# Autodesk Inventor assembly: Drive Roller Assembly 3 (Lexan)
(part 2 of 2)
- Mate:1086: Vex Pro 1x1 rectangular tubing 2 in length:2 ↔ Vex Pro 90 degree gusset (1-8 in):3
- Mate:1087: Spacer 2:4 ↔ Vex Pro 90 degree gusset (1-8 in):3
- Mate:1088: Spacer 2:4 ↔ Vex Pro 90 degree gusset (1-8 in):3
- Mate:1090: Vex Pro 1x1 rectangular tubing 2 in length:4 ↔ Vex Pro 90 degree gusset (1-8 in):4
- Mate:1091: Vex Pro 1x1 rectangular tubing 2 in length:4 ↔ Vex Pro 90 degree gusset (1-8 in):4
- Mate:1092: Vex Pro 1x1 rectangular tubing 14 in length:6 ↔ Vex Pro 90 degree gusset (1-8 in):4
- Mate:1093: Spacer 2:3 ↔ Vex Pro 90 degree gusset (1-8 in):4
- Mate:1094: Spacer 2:6 ↔ Vex Pro 90 degree gusset (1-8 in):4
- Mate:1096: Spacer 2:6 ↔ Vex Pro 90 degree gusset (1-8 in):4
- Mate:1100: Clamp with Piston Assembly:2 ↔ Vex Pro 90 degree gusset (Special) (1-8 in):1
- Mate:1101: Clamp with Piston Assembly:2 ↔ Vex Pro 90 degree gusset (Special) (1-8 in):1
- Mate:1102: Vex Pro 1x1 rectangular tubing 2 in length (Flange Support):2 ↔ Vex Pro 90 degree gusset (Special) (1-8 in):1
- Mate:1103: Pneumatic Piston Front Flange (Rt Custom):2 ↔ Clamp Piston ( 1 in stroke twice, 9-16 bore):1
- Mate:1104: Clamp with Piston Assembly:1 ↔ Vex Pro 90 degree gusset (Special) (1-8 in):2
- Mate:1105: Clamp with Piston Assembly:1 ↔ Vex Pro 90 degree gusset (Special) (1-8 in):2
- Mate:1106: Clamp with Piston Assembly:1 ↔ Vex Pro 90 degree gusset (Special) (1-8 in):2
- Mate:1107: Pneumatic Piston Front Flange (Lt Custom):1 ↔ Clamp Piston ( 1 in stroke twice, 9-16 bore):2
- Mate:1108: Roller End Cap Drive (3-D Printed):5 ↔ Hex Shaft Aluminum 1-2 in (am-2291):2
- Mate:1109: Roller End Cap Drive (3-D Printed):5 ↔ Hex Shaft Aluminum 1-2 in (am-2291):2
- Mate:1110: Roller End Cap Drive (3-D Printed):5 ↔ Hex Shaft Collar 1-2 in (7552K500):23
- Mate:1111: Hex Bearing 1-2 in (FR8ZZ-Hex, am-0279):6 ↔ Hex Shaft Collar 1-2 in (7552K500):23
- Mate:1112: Roller End Cap Drive (3-D Printed):2 ↔ Hex Shaft Collar 1-2 in (7552K500):22
- Mate:1113: Hex Bearing 1-2 in (FR8ZZ-Hex, am-0279):3 ↔ Hex Shaft Collar 1-2 in (7552K500):22
- Flush:30: Roller End Cap Drive (3-D Printed):2 ↔ Hex Shaft Aluminum 1-2 in (am-2291):1
- Mate:1114: Roller End Cap Drive (3-D Printed):2 ↔ Polycarbonate Roller 2 OD 1-16 Thick (8585K64):1
- Mate:1115: Roller End Cap Drive (3-D Printed):2 ↔ Polycarbonate Roller 2 OD 1-16 Thick (8585K64):1
- Mate:1117: Vex Pro 1x1 rectangular tubing 14 in length:6 ↔ Lexan flexible Arm Mount:1
- Mate:1123: Lexan flexible Arm Mount:2 ↔ Hex Shaft Connector (Lexan):1
- Mate:1124: Lexan flexible Arm Mount:2 ↔ Hex Shaft Connector (Lexan):1
- Mate:1125: Lexan flexible Arm Mount:2 ↔ Hex Shaft Connector (Lexan):1
- Mate:1126: Lexan flexible Arm Mount:1 ↔ Hex Shaft Connector (Lexan):2
- Mate:1127: Lexan flexible Arm Mount:1 ↔ Hex Shaft Connector (Lexan):2
- Mate:1128: Lexan flexible Arm Mount:1 ↔ Hex Shaft Connector (Lexan):2
- Mate:1129: Vex Pro 1x1 rectangular tubing 14 in length:6 ↔ Lexan flexible Arm Mount:1
- Mate:1130: Vex Pro 1x1 rectangular tubing 14 in length:6 ↔ Lexan flexible Arm Mount:1
- Mate:1131: Vex Pro 1x1 rectangular tubing 14 in length:6 ↔ Lexan flexible Arm Mount:2
- Mate:1132: Vex Pro 1x1 rectangular tubing 14 in length:6 ↔ Lexan flexible Arm Mount:2
- Mate:1133: Hex Shaft 1-2 in 5 in long (am-0856):1 ↔ Hex Shaft Connector (Lexan):1
- Mate:1134: Hex Shaft Collar 1-2 in (7552K500):30 ↔ Hex Shaft Connector (Lexan):1
- Mate:1135: Hex Shaft 1-2 in 5 in long (am-0856):1 ↔ Hex Shaft Connector (Lexan):2
- Mate:1136: Hex Shaft Collar 1-2 in (7552K500):21 ↔ Hex Shaft Connector (Lexan):2
- [Mate]: Lexan flexible Arm Mount:3 ↔ Hex Shaft Connector (Lexan):3
- [Mate]: Lexan flexible Arm Mount:3 ↔ Hex Shaft Connector (Lexan):3
- [Mate]: Lexan flexible Arm Mount:3 ↔ Hex Shaft Connector (Lexan):3
- Mate:1140: Vex Pro 1x1 rectangular tubing 14 in length:5 ↔ Lexan flexible Arm Mount:3
- Mate:1141: Vex Pro 1x1 rectangular tubing 14 in length:5 ↔ Lexan flexible Arm Mount:3
- [Mate]: Lexan flexible Arm Mount:4 ↔ Hex Shaft Connector (Lexan):4
- [Mate]: Lexan flexible Arm Mount:4 ↔ Hex Shaft Connector (Lexan):4
- [Mate]: Lexan flexible Arm Mount:4 ↔ Hex Shaft Connector (Lexan):4
- Mate:1146: Vex Pro 1x1 rectangular tubing 14 in length:5 ↔ Lexan flexible Arm Mount:4
- Mate:1147: Vex Pro 1x1 rectangular tubing 14 in length:5 ↔ Lexan flexible Arm Mount:4
- Mate:1148: Vex Pro 1x1 rectangular tubing 14 in length:5 ↔ Lexan flexible Arm Mount:4
- Mate:1149: Hex Shaft Collar 1-2 in (7552K500):19 ↔ Hex Shaft Connector (Lexan):4
- Mate:1150: Hex Shaft Collar 1-2 in (7552K500):18 ↔ Hex Shaft Connector (Lexan):3
- Mate:1151: Hex Shaft 1-2 in (am-0856):2 ↔ Hex Shaft Connector (Lexan):4
- Mate:1152: Hex Shaft 1-2 in (am-0856):2 ↔ Hex Shaft Connector (Lexan):4
- Mate:1153 (38.1 mm): Lexan flexible Arm Mount:1 ↔ Lexan flexible Arm Mount:2
- Mate:1154 (38.1 mm): Lexan flexible Arm Mount:3 ↔ Lexan flexible Arm Mount:4
- Flush:31: Hex Shaft 1-2 in (am-0856):2 ↔ Hex Shaft Collar 1-2 in (7552K500):19
## Named parameters: d240_d195 = 0 mm, d241_d196 = 0 mm, d242_d197 = 0 mm, d243_d198 = 0 mm, d305_d302 = 0 mm, d306_d303 = 0 mm, d307_d304 = 0 mm, d334_d317 = 0 mm, d335_d318 = -19.05 mm, d336_d325 = 0 mm, d339_d304 = 0 mm, d343_d308 = 0 mm, d344_d309 = 0 mm, d345_d310 = 0 mm, d346_d316 = 0 mm, d347_d326 = 0 mm, d348_d327 = -7.14375 mm, d349_d328 = 0 mm, d350_d329 = 0 mm, d351_d330 = 0 mm, d352_d331 = 0 mm, d353_d332 = 0 mm, d354_d333 = 0 mm, d770_d743 = 0 mm, d771_d744 = 0 mm, d772_d745 = 0 mm, d773_d746 = 0 mm, d791_d742 = 0 mm, d1331_d1327 = 0 mm, d1332_d1328 = 0 mm, d1398_d1387 = 0 mm, d1399_d1388 = 0 mm, d1400_d1389 = 0 mm, d1404_d1384 = 0 mm, d1405_d1385 = 0 mm, d1406_d1386 = 0 mm
